# Autodesk Inventor assembly: EmergencyWake
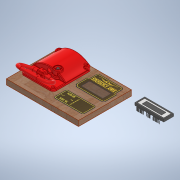
[picture p0: Inventor's stored thumbnail of the model, 180x180]
Saved by Autodesk Inventor 2020 (Build 240168000, 168)
## iProperties
Created: 2020-06-21
Part Number: EmergencyWake
Document SubType Name: Assembly
Designer: Johannes
Author: Johannes
## Documents named in this file (8)
- D:\Dokumente\Projekte\EmergencyWake\CAD\Inventor\EmergencyWake.iam
- D:\Dokumente\Projekte\EmergencyWake\CAD\Inventor\EW_Holzplatte.ipt
- D:\Dokumente\Projekte\EmergencyWake\CAD\Inventor\EW_Display.ipt
- D:\Dokumente\Projekte\EmergencyWake\CAD\Inventor\EW_MessingplatteBedienelemente.ipt
- D:\Dokumente\Projekte\EmergencyWake\CAD\Inventor\EW_MessingplatteUhrzeit.ipt
- D:\Dokumente\Projekte\EmergencyWake\CAD\Inventor\EW_NotbremseGehaeuse.ipt
- D:\Dokumente\Projekte\EmergencyWake\CAD\Inventor\EW_NotbremseHebel.ipt
- D:\Dokumente\Projekte\EmergencyWake\CAD\Inventor\EW_Plexiglas.ipt
## Components (7 placed, 7 different names)
1. EW_Holzplatte:1 — Passend:1, Passend:2, Passend:3, Fluchtend:1, Fluchtend:2, Fluchtend:3, Fluchtend:4, Fluchtend:5, Passend:5, Passend:6, Fluchtend:6
2. EW_Display:1
3. EW_MessingplatteBedienelemente:1 — Passend:2, Fluchtend:5, Passend:4
4. EW_MessingplatteUhrzeit:1 — Passend:3, Fluchtend:3, Fluchtend:4, Passend:4
5. EW_NotbremseGehaeuse:1 — Passend:1, Einfügen:1, Fluchtend:1, Fluchtend:2
6. EW_NotbremseHebel:1 — Einfügen:1
7. EW_Plexiglas:1 — Passend:5, Passend:6, Fluchtend:6
## Relationships (13: Mate 6, Flush 6, Insert 1)
- Passend:1 [Mate]: EW_Holzplatte:1 ↔ EW_NotbremseGehaeuse:1
- Einfügen:1 [Insert] (15 mm): EW_NotbremseGehaeuse:1 ↔ EW_NotbremseHebel:1
- Passend:2 [Mate]: EW_Holzplatte:1 ↔ EW_MessingplatteBedienelemente:1
- Passend:3 [Mate]: EW_Holzplatte:1 ↔ EW_MessingplatteUhrzeit:1
- Fluchtend:1 [Flush] (-10 mm): EW_Holzplatte:1 ↔ EW_NotbremseGehaeuse:1
- Fluchtend:2 [Flush] (-10 mm): EW_Holzplatte:1 ↔ EW_NotbremseGehaeuse:1
- Fluchtend:3 [Flush] (10 mm): EW_Holzplatte:1 ↔ EW_MessingplatteUhrzeit:1
- Fluchtend:4 [Flush] (10 mm): EW_Holzplatte:1 ↔ EW_MessingplatteUhrzeit:1
- Fluchtend:5 [Flush] (10 mm): EW_Holzplatte:1 ↔ EW_MessingplatteBedienelemente:1
- Passend:4 [Mate] (25 mm): EW_MessingplatteBedienelemente:1 ↔ EW_MessingplatteUhrzeit:1
- Passend:5 [Mate]: EW_Holzplatte:1 ↔ EW_Plexiglas:1
- Passend:6 [Mate]: EW_Holzplatte:1 ↔ EW_Plexiglas:1
- Fluchtend:6 [Flush]: EW_Holzplatte:1 ↔ EW_Plexiglas:1
